# Autodesk Inventor assembly: Torque Sensor
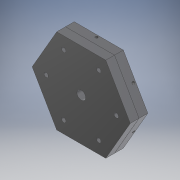
[picture p0: Inventor's stored thumbnail of the model, 180x180]
Saved by Autodesk Inventor 2017 (Build 210142000, 142)
## iProperties
Created: 2018-10-24
Part Number: Torque Sensor
Document SubType Name: Assembly
Designer: Dell
Author: Dell
## Documents named in this file (3)
- C:\Users\Dell\Documents\GitHub\tr2\Torque Sensor\Torque Sensor.iam
- C:\Users\Dell\Documents\GitHub\tr2\Torque Sensor\TS01.ipt
- C:\Users\Dell\Documents\GitHub\tr2\Torque Sensor\TS02.ipt
## Components (2 placed, 2 different names)
1. TS01:1 — Mate:3, Mate:4
2. TS02:1 — Mate:3, Mate:4
## Relationships (2: Mate 2)
- Mate:3: TS01:1 ↔ TS02:1
- Mate:4: TS01:1 ↔ TS02:1
